# Autodesk Inventor assembly: TC-1001
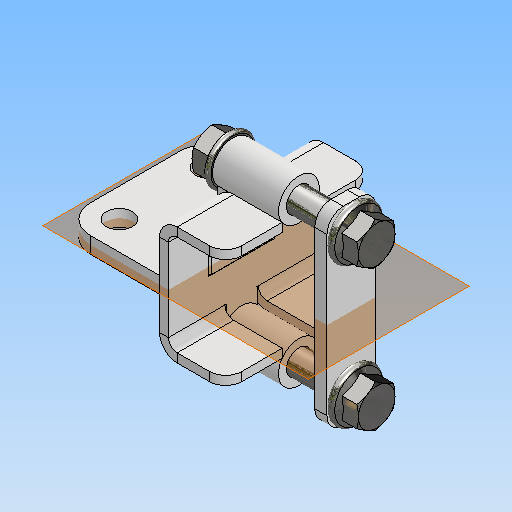
[picture p0: Inventor's stored thumbnail of the model, 512x512]
Saved by Autodesk Inventor 2025.4 (Build 294407000, 407)
## iProperties
Created: 2025-11-28
Part Number: TC-1001
Document SubType Name: Assembly
Designer: josh
Description: 1-1/2" Sq Tube Bolt-on Clamp
Author: josh
## Documents named in this file (7)
- R:\A1- Neuweg Design Data\OM Robotics\CLEANING ROBOT TOWER PROJECT\TC-1001.iam
- R:\A1- Neuweg Design Data\OM Robotics\CLEANING ROBOT TOWER PROJECT\TC-1002.ipt
- R:\A1- Neuweg Design Data\OM Robotics\CLEANING ROBOT TOWER PROJECT\TC-1003.ipt
- R:\A1- Neuweg Design Data\OM Robotics\CLEANING ROBOT TOWER PROJECT\TC-1004.ipt
- R:\A1- Neuweg Design Data\OM Robotics\CLEANING ROBOT TOWER PROJECT\TC-1005.ipt
- C:\Users\Josh\Documents\Inventor\Content Center Files\R2025\en-US\IFI 111\IFI 111 - 3_8-16 UNC x 2.25.ipt
- C:\Users\Josh\Documents\Inventor\Content Center Files\R2025\en-US\IFI (1)\IFI - I0.375 - 16(1).ipt
## Components (9 placed, 6 different names)
1. TC-1005:1 — Flush:10, Flush:11, Flush:12, Insert:1, Insert:2
2. TC-1003:1 — Flush:7, Flush:8, Flush:9, Mate:4
3. TC-1002:1 — Flush:4, Flush:5, Flush:6
4. TC-1004:1 — Flush:1, Flush:2, Flush:3
5. TC-1003:2 — Flush:13, Mate:1, Mate:2, Insert:3
6. Hex Flange Screw - Inch (IFI) 3/8-16 UNC x 2.25:1 — Insert:1, Mate:3
7. Hex Flange Screw - Inch (IFI) 3/8-16 UNC x 2.25:2 — Insert:2
8. Hex Flange Nut - Inch (IFI) I0.375 - 16:1 — Mate:3, Mate:4
9. Hex Flange Nut - Inch (IFI) I0.375 - 16:2 — Insert:3
## Relationships (20: Flush 13, Mate 4, Insert 3)
- Flush:1: TC-1004:1
- Flush:2: TC-1004:1
- Flush:3: TC-1004:1
- Flush:4: TC-1002:1
- Flush:5: TC-1002:1
- Flush:6: TC-1002:1
- Flush:7: TC-1003:1
- Flush:8: TC-1003:1
- Flush:9: TC-1003:1
- Flush:10: TC-1005:1
- Flush:11: TC-1005:1
- Flush:12: TC-1005:1
- Flush:13: TC-1003:2
- Mate:1: TC-1003:2
- Mate:2: TC-1003:2
- Insert:1: TC-1005:1 ↔ Hex Flange Screw - Inch (IFI) 3/8-16 UNC x 2.25:1
- Insert:2: TC-1005:1 ↔ Hex Flange Screw - Inch (IFI) 3/8-16 UNC x 2.25:2
- Mate:3: Hex Flange Screw - Inch (IFI) 3/8-16 UNC x 2.25:1 ↔ Hex Flange Nut - Inch (IFI) I0.375 - 16:1
- Mate:4: TC-1003:1 ↔ Hex Flange Nut - Inch (IFI) I0.375 - 16:1
- Insert:3: TC-1003:2 ↔ Hex Flange Nut - Inch (IFI) I0.375 - 16:2
